# Autodesk Inventor assembly: Actual Robot
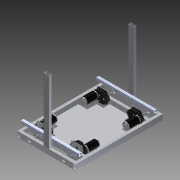
[picture p0: Inventor's stored thumbnail of the model, 180x180]
Saved by Autodesk Inventor 2014 SP1 (Build 180222100, 222)
## iProperties
Created: 2014-01-18
Part Number: Actual Robot
Document SubType Name: Assembly
Designer: Paul
Author: Paul
## Documents named in this file (3)
- C:\FRC_CAD\4859cad\Robot\Actual Robot\Actual Robot.iam
- C:\FRC_CAD\4859cad\Robot\Structure\Frame Assembly\1x1 tube 22in.ipt
- C:\FRC_CAD\4859cad\Robot\Structure\Frame Assembly\2x1 Tube 24in.ipt
## Components (5 placed, 3 different names)
1. FrameAssembly :1 [sub-assembly] — Flush:1, Flush:2, Mate:1, Flush:3, Flush:4, Mate:2, Flush:5, Flush:6
2. 1x1 tube 22in:1 — Flush:1
3. 1x1 tube 22in:2 — Flush:2
4. 2x1 Tube 24in:1 — Mate:1, Flush:3, Flush:5
5. 2x1 Tube 24in:2 — Flush:4, Mate:2, Flush:6
## Relationships (8: Flush 6, Mate 2)
- Flush:1: FrameAssembly :1 ↔ 1x1 tube 22in:1
- Flush:2: FrameAssembly :1 ↔ 1x1 tube 22in:2
- Mate:1: FrameAssembly :1 ↔ 2x1 Tube 24in:1
- Flush:3: FrameAssembly :1 ↔ 2x1 Tube 24in:1
- Flush:4: FrameAssembly :1 ↔ 2x1 Tube 24in:2
- Mate:2: FrameAssembly :1 ↔ 2x1 Tube 24in:2
- Flush:5 (254 mm): FrameAssembly :1 ↔ 2x1 Tube 24in:1
- Flush:6 (254 mm): FrameAssembly :1 ↔ 2x1 Tube 24in:2
